# Autodesk Inventor assembly: gearbox
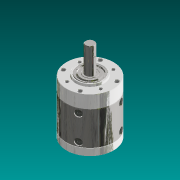
[picture p0: Inventor's stored thumbnail of the model, 180x180]
Saved by Autodesk Inventor 2020.3 (Build 243373000, 373)
## iProperties
Created: 2020-05-14
Part Number: gearbox
Document SubType Name: Assembly
Designer: Svend
Author: Svend
## Documents named in this file (8)
- C:\Users\Svend\OneDrive\Documents\GitHub\BeerMinder\3D-model\gearbox\gearbox.iam
- C:\Users\Svend\OneDrive\Documents\GitHub\BeerMinder\3D-model\bearings\Ball Bearing 608ZZ.ipt
- C:\Users\Svend\OneDrive\Documents\GitHub\BeerMinder\3D-model\gearbox\bovenkantGearbox.ipt
- C:\Users\Svend\OneDrive\Documents\GitHub\BeerMinder\3D-model\gearbox\onderkantGearbox.ipt
- C:\Users\Svend\OneDrive\Documents\GitHub\BeerMinder\3D-model\gearbox\middenGearbox.ipt
- C:\Users\Svend\OneDrive\Documents\GitHub\BeerMinder\3D-model\gearbox\asGearbox.ipt
- C:\Users\Svend\OneDrive\Documents\Inventor\Content Center Files\R2020\en-US\ISO 14581_2013(E)\ISO 14581 - M3x6-4.8.ipt
- C:\Users\Svend\OneDrive\Documents\GitHub\BeerMinder\3D-model\gearbox\spie.ipt
## Components (15 placed, 7 different names)
1. Ball Bearing 608ZZ:1 — Mate:1, Flush:1
2. bovenkantGearbox:1 — Mate:1, Flush:1, Mate:2, Flush:2, Mate:3, Mate:5, Flush:3
3. onderkantGearbox:1 — Mate:4, Mate:6
4. Ball Bearing 608ZZ:2 — Mate:2, Flush:2
5. middenGearbox:1 — Mate:3, Mate:4, Mate:5, Mate:6, Mate:7, Mate:8, Mate:9, Mate:10, Mate:11, Mate:12, Mate:13, Mate:14, Mate:15, Mate:16, Mate:17, Mate:18, Mate:19, Mate:20, Mate:21, Mate:22, Mate:23
6. asGearbox:1 — Mate:7, Flush:3, Mate:24, Mate:25, Mate:26
7. Screw ISO 14581:2013(E) M3x6-4.8:1 — Mate:8, Mate:15
8. Screw ISO 14581:2013(E) M3x6-4.8:2 — Mate:9, Mate:14
9. Screw ISO 14581:2013(E) M3x6-4.8:3 — Mate:20, Mate:23
10. Screw ISO 14581:2013(E) M3x6-4.8:4 — Mate:21, Mate:22
11. Screw ISO 14581:2013(E) M3x6-4.8:5 — Mate:11, Mate:13
12. Screw ISO 14581:2013(E) M3x6-4.8:6 — Mate:16, Mate:18
13. Screw ISO 14581:2013(E) M3x6-4.8:7 — Mate:10, Mate:12
14. Screw ISO 14581:2013(E) M3x6-4.8:8 — Mate:17, Mate:19
15. spie:1 — Mate:24, Mate:25, Mate:26
## Relationships (29: Mate 26, Flush 3)
- Mate:1: Ball Bearing 608ZZ:1 ↔ bovenkantGearbox:1
- Flush:1: Ball Bearing 608ZZ:1 ↔ bovenkantGearbox:1
- Mate:2: bovenkantGearbox:1 ↔ Ball Bearing 608ZZ:2
- Flush:2: bovenkantGearbox:1 ↔ Ball Bearing 608ZZ:2
- Mate:3: bovenkantGearbox:1 ↔ middenGearbox:1
- Mate:4: onderkantGearbox:1 ↔ middenGearbox:1
- Mate:5: bovenkantGearbox:1 ↔ middenGearbox:1
- Mate:6: onderkantGearbox:1 ↔ middenGearbox:1
- Mate:7: middenGearbox:1 ↔ asGearbox:1
- Flush:3 (-23 mm): bovenkantGearbox:1 ↔ asGearbox:1
- Mate:8: middenGearbox:1 ↔ Screw ISO 14581:2013(E) M3x6-4.8:1
- Mate:9: middenGearbox:1 ↔ Screw ISO 14581:2013(E) M3x6-4.8:2
- Mate:10: middenGearbox:1 ↔ Screw ISO 14581:2013(E) M3x6-4.8:7
- Mate:11: middenGearbox:1 ↔ Screw ISO 14581:2013(E) M3x6-4.8:5
- Mate:12: middenGearbox:1 ↔ Screw ISO 14581:2013(E) M3x6-4.8:7
- Mate:13: middenGearbox:1 ↔ Screw ISO 14581:2013(E) M3x6-4.8:5
- Mate:14: middenGearbox:1 ↔ Screw ISO 14581:2013(E) M3x6-4.8:2
- Mate:15: middenGearbox:1 ↔ Screw ISO 14581:2013(E) M3x6-4.8:1
- Mate:16: middenGearbox:1 ↔ Screw ISO 14581:2013(E) M3x6-4.8:6
- Mate:17: middenGearbox:1 ↔ Screw ISO 14581:2013(E) M3x6-4.8:8
- Mate:18: middenGearbox:1 ↔ Screw ISO 14581:2013(E) M3x6-4.8:6
- Mate:19: middenGearbox:1 ↔ Screw ISO 14581:2013(E) M3x6-4.8:8
- Mate:20: middenGearbox:1 ↔ Screw ISO 14581:2013(E) M3x6-4.8:3
- Mate:21: middenGearbox:1 ↔ Screw ISO 14581:2013(E) M3x6-4.8:4
- Mate:22: middenGearbox:1 ↔ Screw ISO 14581:2013(E) M3x6-4.8:4
- Mate:23: middenGearbox:1 ↔ Screw ISO 14581:2013(E) M3x6-4.8:3
- Mate:24: asGearbox:1 ↔ spie:1
- Mate:25: asGearbox:1 ↔ spie:1
- Mate:26: asGearbox:1 ↔ spie:1
